# Autodesk Inventor assembly: Pipette Assembly
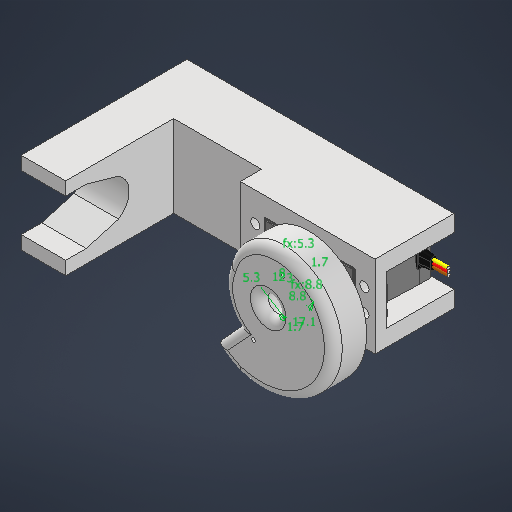
[picture p0: Inventor's stored thumbnail of the model, 512x512]
Saved by Autodesk Inventor 2025.1 (Build 291241000, 241)
## iProperties
Created: 2024-10-19
Part Number: Pipette Assembly
Document SubType Name: Assembly
Designer: 13156
Author: 13156
## Documents named in this file (5)
- C:\Users\jerem\Documents\GitHub\Perovskite-Automated-Synthesis-System\CAD\Pipette\Pipette Assembly.iam
- C:\Users\jerem\Documents\GitHub\Perovskite-Automated-Synthesis-System\CAD\Non 3D Printed Parts\Motors and Servos\Servo MG996R.ipt
- C:\Users\jerem\Documents\GitHub\Perovskite-Automated-Synthesis-System\CAD\Non 3D Printed Parts\Motors and Servos\MG996 2 Arm Pad.ipt
- C:\Users\jerem\Documents\GitHub\Perovskite-Automated-Synthesis-System\CAD\Pipette\Holder2.ipt
- C:\Users\jerem\Documents\GitHub\Perovskite-Automated-Synthesis-System\CAD\Pipette\Cam.ipt
## Components (4 placed, 4 different names)
1. Servo MG996R:1 — Mate:1, Mate:2, Mate:3, Mate:4
2. MG996 2 Arm Pad:1 — Mate:1, Mate:2, Mate:5, Mate:6
3. Holder2:1 — Mate:3, Mate:4
4. Cam:1 — Mate:5, Mate:6
## Relationships (6: Mate 6)
- Mate:1: Servo MG996R:1 ↔ MG996 2 Arm Pad:1
- Mate:2: Servo MG996R:1 ↔ MG996 2 Arm Pad:1
- Mate:3: Servo MG996R:1 ↔ Holder2:1
- Mate:4: Servo MG996R:1 ↔ Holder2:1
- Mate:5: MG996 2 Arm Pad:1 ↔ Cam:1
- Mate:6 (6.762 mm): MG996 2 Arm Pad:1 ↔ Cam:1
